# Autodesk Inventor assembly: wheel with sprocket_MIR
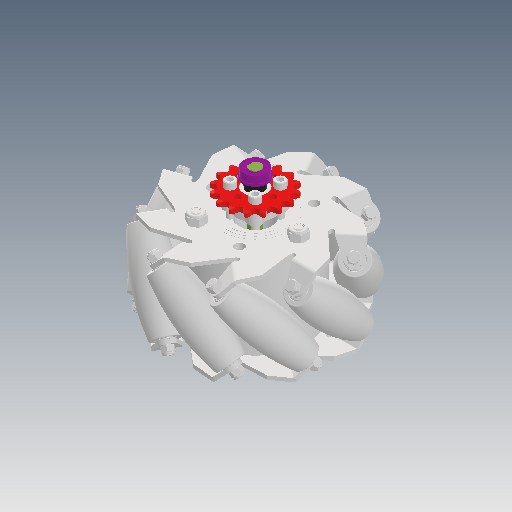
[picture p0: Inventor's stored thumbnail of the model, 512x512]
Saved by Autodesk Inventor 2020 (Build 240168000, 168)
## iProperties
Created: 2019-09-29
Part Number: wheel with sprocket_MIR
Document SubType Name: Assembly
Designer: ball
Author: ball
## Documents named in this file (7)
- C:\FTC\FTC8863CAD\2019 Robot\Mecanum Drive Train\wheel with sprocket_MIR.iam
- C:\FTC\FTC8863CAD\2019 Robot\Mecanum Drive Train\left wheel with clamping hub_MIR.iam
- C:\FTC\FTC8863CAD\Actobotics\615 parts\615102_MIR.ipt
- C:\FTC\FTC8863CAD\Actobotics\535 parts\535198_MIR.ipt
- C:\FTC\FTC8863CAD\Actobotics\633 parts\633104_MIR.ipt
- C:\FTC\FTC8863CAD\2019 Robot\Mecanum Drive Train\3_35 shaft_MIR.ipt
- C:\FTC\FTC8863CAD\StepLibraries\Screws\6-32 x 2_75 SOCKET HEAD CAP SCREW_MIR.ipt
## Components (13 placed, 6 different names)
1. left wheel with clamping hub_MIR:1 [sub-assembly] — Mate:5, Mate:4, Mate:3, Mate:2, Mate:1, Mate:19, Mate:17, Mate:16, Mate:22, Mate:26, Mate:28, Mate:27
2. 615102_MIR:1 — Mate:3, Mate:2, Mate:1, Mate:7, Mate:14, Mate:13, Mate:21, Mate:24, Mate:23, Mate:25
3. 535198_MIR:1 — Mate:19, Mate:18, Flush:1
4. 535198_MIR:2 — Mate:7, Mate:20, Mate:33
5. 633104_MIR:1 — Mate:18, Mate:17, Mate:16
6. 633104_MIR:2 — Mate:14, Mate:13, Mate:30
7. 3_35 shaft_MIR:1 — Flush:1, Mate:20, Mate:29, Mate:31
8. 6-32 x 2_75 SOCKET HEAD CAP SCREW_MIR:1 — Mate:22, Mate:21
9. 6-32 x 2_75 SOCKET HEAD CAP SCREW_MIR:2 — Mate:26, Mate:24
10. 6-32 x 2_75 SOCKET HEAD CAP SCREW_MIR:3 — Mate:28, Mate:23
11. 6-32 x 2_75 SOCKET HEAD CAP SCREW_MIR:4 — Mate:27, Mate:25
12. 633104_MIR:3 — Mate:30, Mate:29, Mate:32
13. 633104_MIR:4 — Mate:33, Mate:32, Mate:31
## Relationships (27: Mate 26, Flush 1)
- Mate:5: left wheel with clamping hub_MIR:1
- Mate:4: left wheel with clamping hub_MIR:1
- Mate:3: left wheel with clamping hub_MIR:1 ↔ 615102_MIR:1
- Mate:2: left wheel with clamping hub_MIR:1 ↔ 615102_MIR:1
- Mate:1: left wheel with clamping hub_MIR:1 ↔ 615102_MIR:1
- Mate:19: left wheel with clamping hub_MIR:1 ↔ 535198_MIR:1
- Mate:7: 615102_MIR:1 ↔ 535198_MIR:2
- Mate:18: 535198_MIR:1 ↔ 633104_MIR:1
- Mate:17: left wheel with clamping hub_MIR:1 ↔ 633104_MIR:1
- Mate:16: left wheel with clamping hub_MIR:1 ↔ 633104_MIR:1
- Mate:14: 615102_MIR:1 ↔ 633104_MIR:2
- Mate:13: 615102_MIR:1 ↔ 633104_MIR:2
- Flush:1: 535198_MIR:1 ↔ 3_35 shaft_MIR:1
- Mate:20: 535198_MIR:2 ↔ 3_35 shaft_MIR:1
- Mate:22: left wheel with clamping hub_MIR:1 ↔ 6-32 x 2_75 SOCKET HEAD CAP SCREW_MIR:1
- Mate:21: 615102_MIR:1 ↔ 6-32 x 2_75 SOCKET HEAD CAP SCREW_MIR:1
- Mate:26: left wheel with clamping hub_MIR:1 ↔ 6-32 x 2_75 SOCKET HEAD CAP SCREW_MIR:2
- Mate:24: 615102_MIR:1 ↔ 6-32 x 2_75 SOCKET HEAD CAP SCREW_MIR:2
- Mate:28: left wheel with clamping hub_MIR:1 ↔ 6-32 x 2_75 SOCKET HEAD CAP SCREW_MIR:3
- Mate:23: 615102_MIR:1 ↔ 6-32 x 2_75 SOCKET HEAD CAP SCREW_MIR:3
- Mate:27: left wheel with clamping hub_MIR:1 ↔ 6-32 x 2_75 SOCKET HEAD CAP SCREW_MIR:4
- Mate:25: 615102_MIR:1 ↔ 6-32 x 2_75 SOCKET HEAD CAP SCREW_MIR:4
- Mate:30: 633104_MIR:2 ↔ 633104_MIR:3
- Mate:29: 3_35 shaft_MIR:1 ↔ 633104_MIR:3
- Mate:33: 535198_MIR:2 ↔ 633104_MIR:4
- Mate:32: 633104_MIR:3 ↔ 633104_MIR:4
- Mate:31: 3_35 shaft_MIR:1 ↔ 633104_MIR:4
